# Autodesk Inventor assembly: Assembly_for_al_2l
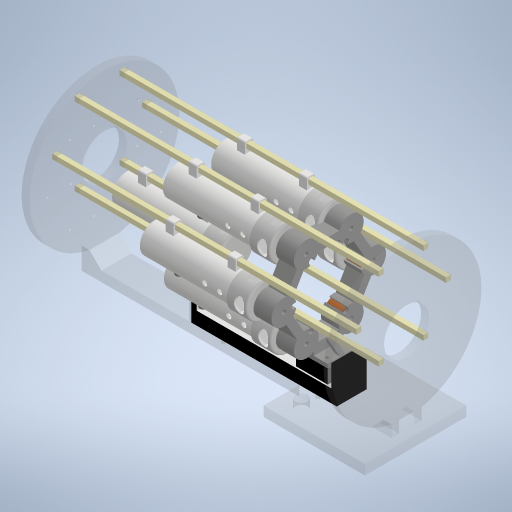
[picture p0: Inventor's stored thumbnail of the model, 512x512]
Saved by Autodesk Inventor 2023 (Build 270158000, 158)
## iProperties
Created: 2022-11-03
Part Number: Assembly_for_al_2l
Document SubType Name: Assembly
Designer: Admin
Author: Admin
## Documents named in this file (9)
- D:\multimate\Mouse_restrainer_V3\Assembly_for_al_2l.iam
- D:\multimate\Mouse_restrainer_V3\base2.ipt
- D:\multimate\Mouse_restrainer_V3\linear trail.ipt
- D:\multimate\Mouse_restrainer_V3\motor on trail.ipt
- D:\multimate\Mouse_restrainer_V3\support_electrical_magnets.ipt
- D:\multimate\Mouse_restrainer_V3\stock.ipt
- D:\multimate\Mouse_restrainer_V3\electromagnet.ipt
- D:\multimate\Mouse_restrainer_V3\restrainer.iam
- D:\multimate\Mouse_restrainer_V3\micro_magnets_2mm1mm.ipt
## Components (24 placed, 8 different names)
1. base2:1 — Rigid:1, Rigid:3, Rigid:11, Rigid:12, Rigid:13, Rigid:14, Rigid:15
2. linear trail:1 — Rigid:1, Cylindrical:1, Angle:1
3. motor on trail:1 — Cylindrical:1, Angle:1, Rigid:2
4. support_electrical_magnets:1 — Rigid:2, Rotational:1, Rotational:2, Rotational:3, Rotational:4, Rotational:5, Rotational:6
5. stock:1 — Slider:2, Rigid:14
6. stock:2 — Slider:3, Rigid:13
7. stock:3 — Rigid:3, Slider:6
8. stock:4 — Slider:1, Rigid:12
9. stock:5 — Slider:5, Rigid:11
10. stock:6 — Slider:4, Rigid:15
11. electromagnet:1 — Rotational:5
12. electromagnet:2 — Rotational:1
13. electromagnet:3 — Rotational:6
14. electromagnet:4 — Rotational:3
15. electromagnet:5 — Rotational:4
16. electromagnet:6 — Rotational:2
17. restrainer:1 [sub-assembly] — Slider:1
18. restrainer:2 [sub-assembly] — Slider:6, Rotational:7, Rotational:8
19. restrainer:3 [sub-assembly] — Slider:2
20. restrainer:4 [sub-assembly] — Slider:3
21. restrainer:5 [sub-assembly] — Slider:4
22. restrainer:6 [sub-assembly] — Slider:5
23. micro_magnets_2mm1mm:1 — Rotational:7
24. micro_magnets_2mm1mm:2 — Rotational:8
## Relationships (24: WeldJoint 8, RevoluteJoint 8, TranslationJoint 6, CylindricalJoint 1, Angle 1)
- Rigid:1 [WeldJoint]: base2:1 ↔ linear trail:1
- Cylindrical:1: linear trail:1 ↔ motor on trail:1
- Angle:1 (0 deg): linear trail:1 ↔ motor on trail:1
- Rigid:2 [WeldJoint]: motor on trail:1 ↔ support_electrical_magnets:1
- Rigid:3 [WeldJoint]: base2:1 ↔ stock:3
- Rotational:1 [RevoluteJoint]: support_electrical_magnets:1 ↔ electromagnet:2
- Rotational:2 [RevoluteJoint]: support_electrical_magnets:1 ↔ electromagnet:6
- Rotational:3 [RevoluteJoint]: support_electrical_magnets:1 ↔ electromagnet:4
- Rotational:4 [RevoluteJoint]: support_electrical_magnets:1 ↔ electromagnet:5
- Rotational:5 [RevoluteJoint]: support_electrical_magnets:1 ↔ electromagnet:1
- Rotational:6 [RevoluteJoint]: support_electrical_magnets:1 ↔ electromagnet:3
- Slider:1 [TranslationJoint]: stock:4 ↔ restrainer:1
- Slider:2 [TranslationJoint]: stock:1 ↔ restrainer:3
- Slider:3 [TranslationJoint]: stock:2 ↔ restrainer:4
- Slider:4 [TranslationJoint]: stock:6 ↔ restrainer:5
- Slider:5 [TranslationJoint]: stock:5 ↔ restrainer:6
- Slider:6 [TranslationJoint]: stock:3 ↔ restrainer:2
- Rigid:11 [WeldJoint]: base2:1 ↔ stock:5
- Rigid:12 [WeldJoint]: base2:1 ↔ stock:4
- Rigid:13 [WeldJoint]: base2:1 ↔ stock:2
- Rigid:14 [WeldJoint]: base2:1 ↔ stock:1
- Rigid:15 [WeldJoint]: base2:1 ↔ stock:6
- Rotational:7 [RevoluteJoint]: restrainer:2 ↔ micro_magnets_2mm1mm:1
- Rotational:8 [RevoluteJoint]: restrainer:2 ↔ micro_magnets_2mm1mm:2
